# Autodesk Inventor assembly: FullV3
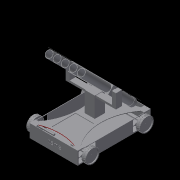
[picture p0: Inventor's stored thumbnail of the model, 180x180]
Saved by Autodesk Inventor 2019 (Build 230136000, 136)
## iProperties
Created: 2021-09-16
Part Number: FullV3
Document SubType Name: Assembly
Designer: timmy
Author: timmy
## Documents named in this file (9)
- S:\Inventor\RoboCatz\T-Shirt\FullV3.iam
- S:\Inventor\RoboCatz\T-Shirt\NamePlateV1.ipt
- S:\Inventor\RoboCatz\T-Shirt\R-O-SideV1.ipt
- S:\Inventor\RoboCatz\T-Shirt\LauncherFullV1.iam
- S:\Inventor\RoboCatz\T-Shirt\BottomV1.ipt
- S:\Inventor\RoboCatz\T-Shirt\AxleBearingV1.ipt
- S:\Inventor\RoboCatz\T-Shirt\6x10inAxleV1.ipt
- S:\Inventor\RoboCatz\T-Shirt\TopV3.ipt
- S:\Inventor\RoboCatz\T-Shirt\WheelV2.ipt
## Components (19 placed, 8 different names)
1. NamePlateV1:1 — Mate:1, Flush:2, Flush:3, Flush:4, Flush:5, Flush:6, Flush:14, Flush:42, Flush:43
2. R-O-SideV1:1 — Flush:4, Flush:5, Flush:6, Mate:6, Mate:30, Mate:31, Mate:36, Mate:37
3. NamePlateV1:2 — Flush:7, Flush:8, Flush:9
4. R-O-SideV1:2 — Mate:1, Flush:2, Flush:3, Flush:7, Flush:8, Flush:9, Mate:2, Angle:1, Mate:3, Angle:3, Mate:17, Flush:15, Mate:18, Mate:19, Mate:24, Mate:25, Flush:44
5. LauncherFullV1:1 [sub-assembly] — Mate:55, Mate:56, Mate:57
6. BottomV1:1 — Flush:14, Mate:17, Flush:15
7. AxleBearingV1:1 — Mate:30, Mate:31, Flush:20, Mate:32, Mate:33
8. AxleBearingV1:2 — Mate:36, Mate:37, Flush:36, Mate:38, Mate:39
9. AxleBearingV1:3 — Mate:24, Mate:25, Flush:18, Mate:26, Mate:27
10. AxleBearingV1:4 — Mate:18, Mate:19, Mate:20, Flush:16, Mate:21
11. 6x10inAxleV1:1 — Mate:20, Flush:16, Mate:21, Flush:48, Mate:49, Mate:50
12. 6x10inAxleV1:2 — Flush:36, Mate:38, Mate:39, Flush:49, Mate:51, Mate:52
13. 6x10inAxleV1:3 — Flush:20, Mate:32, Mate:33, Flush:50, Mate:53, Mate:54
14. 6x10inAxleV1:4 — Flush:18, Mate:26, Mate:27, Flush:47, Mate:47, Mate:48
15. TopV3:1 — Flush:42, Flush:43, Flush:44, Mate:55, Mate:56, Mate:57
16. WheelV2:1 — Flush:47, Mate:47, Mate:48
17. WheelV2:2 — Flush:48, Mate:49, Mate:50
18. WheelV2:3 — Flush:50, Mate:53, Mate:54
19. WheelV2:4 — Flush:49, Mate:51, Mate:52
## Relationships (56: Mate 32, Flush 21, Angle 3)
- Mate:1: NamePlateV1:1 ↔ R-O-SideV1:2
- Flush:2: NamePlateV1:1 ↔ R-O-SideV1:2
- Flush:3: NamePlateV1:1 ↔ R-O-SideV1:2
- Flush:4: NamePlateV1:1 ↔ R-O-SideV1:1
- Flush:5: NamePlateV1:1 ↔ R-O-SideV1:1
- Flush:6: NamePlateV1:1 ↔ R-O-SideV1:1
- Flush:7: NamePlateV1:2 ↔ R-O-SideV1:2
- Flush:8: NamePlateV1:2 ↔ R-O-SideV1:2
- Flush:9: NamePlateV1:2 ↔ R-O-SideV1:2
- Mate:2: R-O-SideV1:2
- Angle:1 (45 deg): R-O-SideV1:2
- Mate:3: R-O-SideV1:2
- Angle:2 (90 deg)
- Mate:6: R-O-SideV1:1
- Angle:3 (135 deg): R-O-SideV1:2
- Flush:14: NamePlateV1:1 ↔ BottomV1:1
- Mate:17: R-O-SideV1:2 ↔ BottomV1:1
- Flush:15: R-O-SideV1:2 ↔ BottomV1:1
- Mate:18: R-O-SideV1:2 ↔ AxleBearingV1:4
- Mate:19: R-O-SideV1:2 ↔ AxleBearingV1:4
- Mate:20: AxleBearingV1:4 ↔ 6x10inAxleV1:1
- Flush:16 (50.8 mm): AxleBearingV1:4 ↔ 6x10inAxleV1:1
- Mate:21: AxleBearingV1:4 ↔ 6x10inAxleV1:1
- Mate:24: R-O-SideV1:2 ↔ AxleBearingV1:3
- Mate:25: R-O-SideV1:2 ↔ AxleBearingV1:3
- Flush:18 (50.8 mm): AxleBearingV1:3 ↔ 6x10inAxleV1:4
- Mate:26: AxleBearingV1:3 ↔ 6x10inAxleV1:4
- Mate:27: AxleBearingV1:3 ↔ 6x10inAxleV1:4
- Mate:30: R-O-SideV1:1 ↔ AxleBearingV1:1
- Mate:31: R-O-SideV1:1 ↔ AxleBearingV1:1
- Flush:20 (50.8 mm): AxleBearingV1:1 ↔ 6x10inAxleV1:3
- Mate:32: AxleBearingV1:1 ↔ 6x10inAxleV1:3
- Mate:33: AxleBearingV1:1 ↔ 6x10inAxleV1:3
- Mate:36: R-O-SideV1:1 ↔ AxleBearingV1:2
- Mate:37: R-O-SideV1:1 ↔ AxleBearingV1:2
- Flush:36 (-50.8 mm): AxleBearingV1:2 ↔ 6x10inAxleV1:2
- Mate:38: AxleBearingV1:2 ↔ 6x10inAxleV1:2
- Mate:39: AxleBearingV1:2 ↔ 6x10inAxleV1:2
- Flush:42: NamePlateV1:1 ↔ TopV3:1
- Flush:43: NamePlateV1:1 ↔ TopV3:1
- Flush:44: R-O-SideV1:2 ↔ TopV3:1
- Flush:47: 6x10inAxleV1:4 ↔ WheelV2:1
- Mate:47: 6x10inAxleV1:4 ↔ WheelV2:1
- Mate:48: 6x10inAxleV1:4 ↔ WheelV2:1
- Flush:48: 6x10inAxleV1:1 ↔ WheelV2:2
- Mate:49: 6x10inAxleV1:1 ↔ WheelV2:2
- Mate:50: 6x10inAxleV1:1 ↔ WheelV2:2
- Flush:49: 6x10inAxleV1:2 ↔ WheelV2:4
- Mate:51: 6x10inAxleV1:2 ↔ WheelV2:4
- Mate:52: 6x10inAxleV1:2 ↔ WheelV2:4
- Flush:50: 6x10inAxleV1:3 ↔ WheelV2:3
- Mate:53: 6x10inAxleV1:3 ↔ WheelV2:3
- Mate:54: 6x10inAxleV1:3 ↔ WheelV2:3
- Mate:55: LauncherFullV1:1 ↔ TopV3:1
- Mate:56: LauncherFullV1:1 ↔ TopV3:1
- Mate:57: LauncherFullV1:1 ↔ TopV3:1
